# Autodesk Inventor assembly: 3030_T_connector_assembled
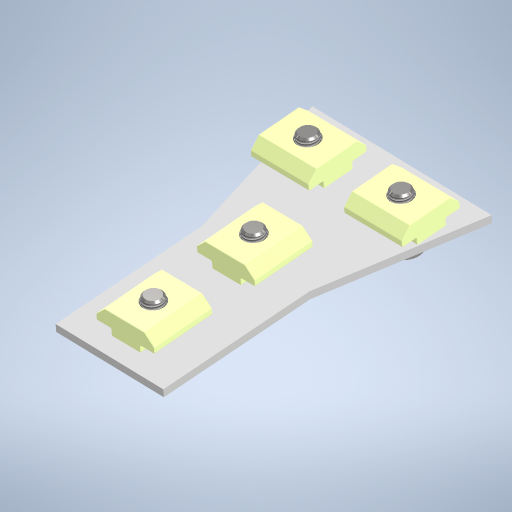
[picture p0: Inventor's stored thumbnail of the model, 512x512]
Saved by Autodesk Inventor 2024 (Build 280153000, 153)
## iProperties
Created: 2025-12-08
Part Number: 3030_T_connector_assembled
Document SubType Name: Assembly
Designer: schar
Author: schar
## Documents named in this file (4)
- C:\Users\schar\Desktop\projectBlueprint\AMSTS\hardware\3030_T_connector_assembled.iam
- C:\Users\schar\Desktop\projectBlueprint\AMSTS\hardware\ConnectTx3030_m6.ipt
- C:\Users\schar\Desktop\projectBlueprint\AMSTS\hardware\3030_tnut_m6.ipt
- C:\Users\schar\Documents\Inventor\Content Center Files\R2024\en-US\AS 1420\AS 1420 - 1973 - M5 x 10.ipt
## Components (9 placed, 3 different names)
1. ConnectTx3030_m6:1 — Mate:1, Mate:2, Mate:3, Mate:4, Mate:10, Mate:12, Mate:13, Mate:15
2. AS 1420 - Metric M5 x 10:1 — Mate:4, Mate:16
3. AS 1420 - Metric M5 x 10:2 — Mate:3, Mate:14
4. AS 1420 - Metric M5 x 10:3 — Mate:2, Mate:11
5. AS 1420 - Metric M5 x 10:4 — Mate:1, Mate:9
6. 3030_tnut_m6:3 — Mate:9, Mate:10
7. 3030_tnut_m6:4 — Mate:11, Mate:12
8. 3030_tnut_m6:5 — Mate:13, Mate:14
9. 3030_tnut_m6:6 — Mate:15, Mate:16
## Relationships (12: Mate 12)
- Mate:1: ConnectTx3030_m6:1 ↔ AS 1420 - Metric M5 x 10:4
- Mate:2: ConnectTx3030_m6:1 ↔ AS 1420 - Metric M5 x 10:3
- Mate:3: ConnectTx3030_m6:1 ↔ AS 1420 - Metric M5 x 10:2
- Mate:4: ConnectTx3030_m6:1 ↔ AS 1420 - Metric M5 x 10:1
- Mate:9: AS 1420 - Metric M5 x 10:4 ↔ 3030_tnut_m6:3
- Mate:10 (0.357 mm): ConnectTx3030_m6:1 ↔ 3030_tnut_m6:3
- Mate:11: AS 1420 - Metric M5 x 10:3 ↔ 3030_tnut_m6:4
- Mate:12 (0.367 mm): ConnectTx3030_m6:1 ↔ 3030_tnut_m6:4
- Mate:13 (0.357 mm): ConnectTx3030_m6:1 ↔ 3030_tnut_m6:5
- Mate:14: AS 1420 - Metric M5 x 10:2 ↔ 3030_tnut_m6:5
- Mate:15 (0.357 mm): ConnectTx3030_m6:1 ↔ 3030_tnut_m6:6
- Mate:16: AS 1420 - Metric M5 x 10:1 ↔ 3030_tnut_m6:6
